# Autodesk Inventor assembly: Motor_Section
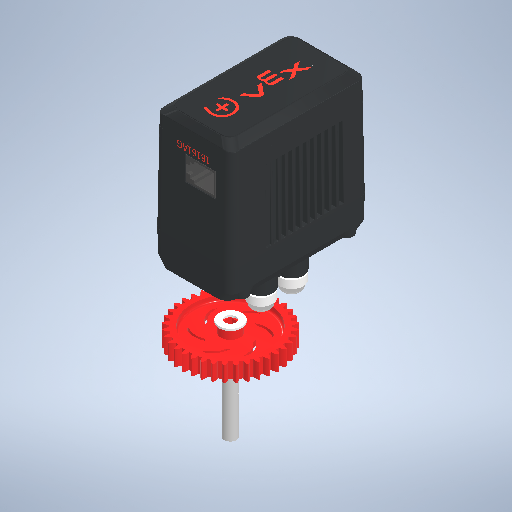
[picture p0: Inventor's stored thumbnail of the model, 512x512]
Saved by Autodesk Inventor 2025 (Build 290162000, 162)
## iProperties
Created: 2024-12-08
Part Number: Motor_Section
Document SubType Name: Assembly
Designer: Aditya Koduri
Author: Aditya Koduri
## Documents named in this file (10)
- C:\Users\mzart\Downloads\Full_Cad_Model\Motor_Section.iam
- C:\Users\mzart\Downloads\VEX-CAD-Inventor-main\VEX-CAD-Inventor-main\Motion\Spacers\Washer Teflon\TWasher .375 OD x .03125.ipt
- C:\Users\mzart\Downloads\VEX-CAD-Inventor-main\VEX-CAD-Inventor-main\Motion\Gears\LS 36T Gear.ipt
- C:\Users\mzart\Downloads\Full_Cad_Model\Thin_spacer_custom.ipt
- C:\Users\mzart\Downloads\VEX-CAD-Inventor-main\VEX-CAD-Inventor-main\Electronics\V5 Motor.ipt
- C:\Users\mzart\Downloads\VEX-CAD-Inventor-main\VEX-CAD-Inventor-main\Motion\Spacers\Spacer Nylon .313 OD\NSpacer .313 OD x .125.ipt
- C:\Users\mzart\Downloads\VEX-CAD-Inventor-main\VEX-CAD-Inventor-main\Structure\Hardware\Screw Steel - Hex\SScrew Hex Smooth .500.ipt
- C:\Users\mzart\Downloads\VEX-CAD-Inventor-main\VEX-CAD-Inventor-main\Motion\Spacers\Washer Teflon.ipt
- C:\Users\mzart\Downloads\VEX-CAD-Inventor-main\VEX-CAD-Inventor-main\Motion\Spacers\Spacer Nylon .313 OD.ipt
- C:\Users\mzart\Downloads\VEX-CAD-Inventor-main\VEX-CAD-Inventor-main\Structure\Hardware\Screw Steel - Hex.ipt
## Components (11 placed, 6 different names)
1. TWasher .375 OD x .03125:1
2. LS 36T Gear:1
3. Thin_spacer_custom:1
4. Thin_spacer_custom:2
5. Thin_spacer_custom:3
6. Thin_spacer_custom:4
7. V5 Motor:1
8. NSpacer .313 OD x .125:1
9. NSpacer .313 OD x .125:2
10. SScrew Hex Smooth .500:1
11. SScrew Hex Smooth .500:2
## Relationships (7: Insert 7)
- [Insert]: TWasher .375 OD x .03125:1 ↔ LS 36T Gear:1
- [Insert]: Thin_spacer_custom:1 ↔ Thin_spacer_custom:3
- [Insert]: Thin_spacer_custom:1 ↔ Thin_spacer_custom:4
- [Insert]: Thin_spacer_custom:2 ↔ Thin_spacer_custom:3
- [Insert]: LS 36T Gear:1 ↔ Thin_spacer_custom:2
- [Insert]: V5 Motor:1 ↔ NSpacer .313 OD x .125:1
- [Insert]: V5 Motor:1 ↔ NSpacer .313 OD x .125:2
